# Autodesk Inventor assembly: SRM with Smoke Grain
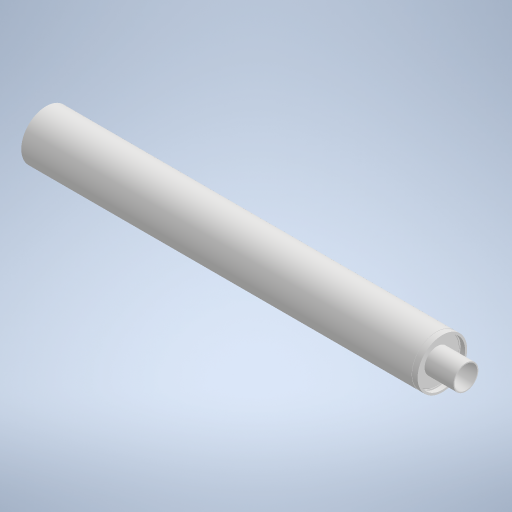
[picture p0: Inventor's stored thumbnail of the model, 512x512]
Saved by Autodesk Inventor 2024 (Build 280153000, 153)
## iProperties
Created: 2024-01-11
Part Number: SRM with Smoke Grain
Document SubType Name: Assembly
Designer: auror
Author: auror
## Documents named in this file (8)
- C:\Users\auror\Documents\TU Delft\DARE\Git\Scrambler-2-CAD\Autodesk\SRM with Smoke Grain.iam
- C:\Users\auror\Documents\TU Delft\DARE\Git\Scrambler-2-CAD\Autodesk\Grain.ipt
- C:\Users\auror\Documents\TU Delft\DARE\Git\Scrambler-2-CAD\Autodesk\Spacer_ring.ipt
- C:\Users\auror\Documents\TU Delft\DARE\Git\Scrambler-2-CAD\Autodesk\Smoke grain.ipt
- C:\Users\auror\Documents\TU Delft\DARE\Git\Scrambler-2-CAD\Autodesk\SRM 2020 Casing EE5.ipt
- SRM 2020 Casing EE5.ipt
- C:\Users\auror\Documents\TU Delft\DARE\Git\Scrambler-2-CAD\Autodesk\Nozzle.ipt
- C:\Users\auror\Documents\TU Delft\DARE\Git\Scrambler-2-CAD\Autodesk\Endcap.ipt
## Components (14 placed, 6 different names)
1. Grain:1 — Mate:35, Mate:36, Mate:37, Mate:38
2. Grain:2 — Mate:43, Mate:44, Mate:45, Mate:46
3. Grain:3 — Mate:30, Mate:31, Mate:33, Mate:34
4. Grain:4 — Mate:39, Mate:40, Mate:41, Mate:42, Mate:44
5. Spacer_ring:1 — Mate:33, Mate:34, Mate:35, Mate:36
6. Spacer_ring:2 — Mate:41, Mate:42, Mate:43
7. Spacer_ring:3 — Mate:45, Mate:46
8. Spacer_ring:4 — Mate:37, Mate:38, Mate:39, Mate:40
9. Spacer_ring:5 — Mate:47, Mate:48, Mate:49
10. Smoke grain:1 — Mate:25, Mate:28, Mate:29, Mate:47, Mate:48
11. Spacer_ring:6 — Mate:28, Mate:29, Mate:30, Mate:31
12. SRM 2020 Casing EE5:1 — Mate:22, Mate:26, Mate:27
13. Nozzle:1 — Mate:22, Mate:27
14. Endcap:1 — Mate:25, Mate:26, Mate:49
## Relationships (25: Mate 25)
- Mate:22: SRM 2020 Casing EE5:1 ↔ Nozzle:1
- Mate:25: Smoke grain:1 ↔ Endcap:1
- Mate:26: SRM 2020 Casing EE5:1 ↔ Endcap:1
- Mate:27: SRM 2020 Casing EE5:1 ↔ Nozzle:1
- Mate:28: Smoke grain:1 ↔ Spacer_ring:6
- Mate:29: Smoke grain:1 ↔ Spacer_ring:6
- Mate:30: Grain:3 ↔ Spacer_ring:6
- Mate:31: Grain:3 ↔ Spacer_ring:6
- Mate:33: Grain:3 ↔ Spacer_ring:1
- Mate:34: Grain:3 ↔ Spacer_ring:1
- Mate:35: Grain:1 ↔ Spacer_ring:1
- Mate:36: Grain:1 ↔ Spacer_ring:1
- Mate:37: Grain:1 ↔ Spacer_ring:4
- Mate:38: Grain:1 ↔ Spacer_ring:4
- Mate:39: Grain:4 ↔ Spacer_ring:4
- Mate:40: Grain:4 ↔ Spacer_ring:4
- Mate:41: Grain:4 ↔ Spacer_ring:2
- Mate:42: Grain:4 ↔ Spacer_ring:2
- Mate:43: Grain:2 ↔ Spacer_ring:2
- Mate:44: Grain:2 ↔ Grain:4
- Mate:45: Grain:2 ↔ Spacer_ring:3
- Mate:46: Grain:2 ↔ Spacer_ring:3
- Mate:47: Spacer_ring:5 ↔ Smoke grain:1
- Mate:48: Spacer_ring:5 ↔ Smoke grain:1
- Mate:49: Spacer_ring:5 ↔ Endcap:1
